# Autodesk Inventor assembly: s-assy-pulley-j4
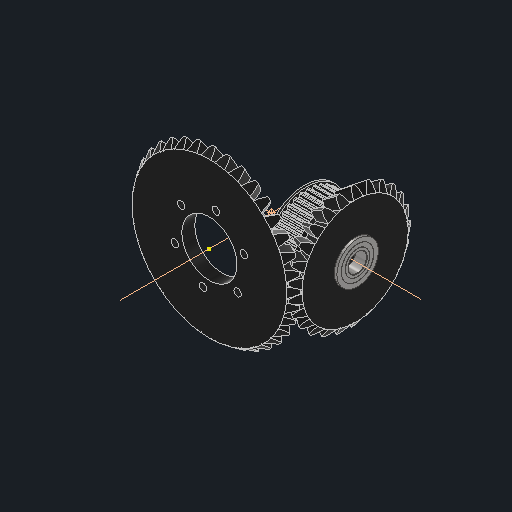
[picture p0: Inventor's stored thumbnail of the model, 512x512]
Saved by Autodesk Inventor 2022 (Build 260153000, 153)
## iProperties
Created: 2021-07-25
Part Number: s-assy-pulley-j4
Document SubType Name: Assembly
Designer: yuto6
Mass: 52.2344 g
Surface Area: 203.948 cm^2
Volume: 39.2193 cm^3
Density: 1.33185 g/cm^3
Author: yuto6
## Documents named in this file (3)
- C:\Users\yuta0\Documents\GitHub\catchrobo_hardware\assy-robot\s-assy-pulley-j4.iam
- C:\Users\yuta0\Documents\GitHub\catchrobo_hardware\assy-robot\FL688ZZ.ipt
- C:\Users\yuta0\Documents\GitHub\catchrobo_hardware\assy-robot\かさ歯車18.iam
## Components (3 placed, 2 different names)
1. FL688ZZ:1 — メイト:2, メイト:8
2. かさ歯車:1 [sub-assembly] — メイト:2, メイト:4, メイト:5, メイト:6, メイト:7, メイト:8
3. FL688ZZ:2 — メイト:4, メイト:7
## Relationships (6: Mate 6)
- メイト:2 [Mate]: FL688ZZ:1 ↔ かさ歯車:1
- メイト:4 [Mate]: かさ歯車:1 ↔ FL688ZZ:2
- メイト:5 [Mate]: かさ歯車:1
- メイト:6 [Mate]: かさ歯車:1
- メイト:7 [Mate]: かさ歯車:1 ↔ FL688ZZ:2
- メイト:8 [Mate]: FL688ZZ:1 ↔ かさ歯車:1
